# Autodesk Inventor assembly: FullUnitMockup
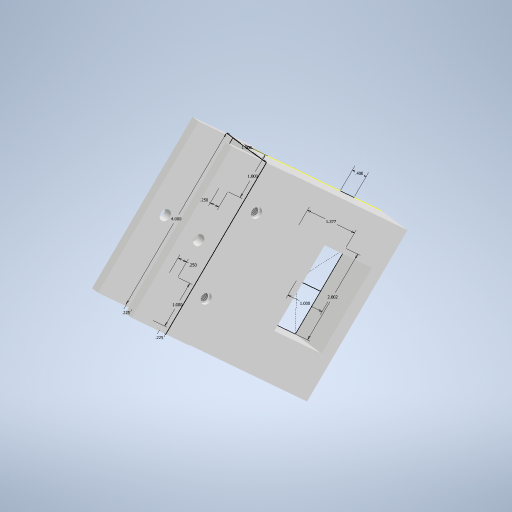
[picture p0: Inventor's stored thumbnail of the model, 512x512]
Saved by Autodesk Inventor 2024.1 (Build 281209000, 209)
## iProperties
Created: 2024-08-21
Part Number: FullUnitMockup
Document SubType Name: Assembly
Designer: pab2
Author: pab2
## Documents named in this file (3)
- C:\Users\pab2\Documents\GitHub\AFL-hardware-devel\Instrument-Interfacing\SANS ThermalBlock\FullUnitMockup.iam
- C:\Users\pab2\Documents\GitHub\AFL-hardware-devel\Instrument-Interfacing\SANS ThermalBlock\Al thermal core.ipt
- C:\Users\pab2\Documents\GitHub\AFL-hardware-devel\Instrument-Interfacing\SANS ThermalBlock\Rail Clip.ipt
## Components (2 placed, 2 different names)
1. Al thermal core:1 — Mate:1, Mate:2
2. Rail Clip:1 — Mate:1, Mate:2
## Relationships (2: Mate 2)
- Mate:1: Al thermal core:1 ↔ Rail Clip:1
- Mate:2: Al thermal core:1 ↔ Rail Clip:1
